# Autodesk Inventor assembly: KegelWelle3.ipt
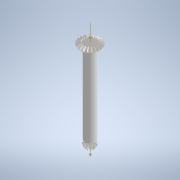
[picture p0: Inventor's stored thumbnail of the model, 180x180]
Saved by Autodesk Inventor 2021 (Build 250183000, 183)
## iProperties
Created: 2021-01-29
Part Number: KegelWelle3.ipt
Document SubType Name: Assembly
Designer: LETPJG
Author: LETPJG
## Documents named in this file (4)
- C:\Users\LETPJG\Documents\Vault\Gruppen\Gruppe 2\Entwurf\Amphibienfahrzeug\KegelWelle3.ipt.iam
- C:\Users\LETPJG\Documents\Vault\Gruppen\Gruppe 2\Entwurf\Amphibienfahrzeug\Planeten\Konstruktions-Assistent\Kegelrad22.ipt
- C:\Users\LETPJG\Documents\Vault\Gruppen\Gruppe 2\Entwurf\Amphibienfahrzeug\Planeten\Konstruktions-Assistent\Kegelrad12.ipt
- C:\Users\LETPJG\Documents\Vault\Gruppen\Gruppe 2\Entwurf\Amphibienfahrzeug\BauteilWelle7.ipt
## Components (3 placed, 3 different names)
1. Kegelrad2:1 — Einfügen:2
2. Kegelrad1:1 — Einfügen:1
3. BauteilWelle7:1 — Einfügen:1, Einfügen:2
## Relationships (2: Insert 2)
- Einfügen:1 [Insert]: Kegelrad1:1 ↔ BauteilWelle7:1
- Einfügen:2 [Insert]: Kegelrad2:1 ↔ BauteilWelle7:1
